# Autodesk Inventor assembly: boltAssembly
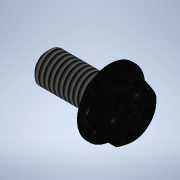
[picture p0: Inventor's stored thumbnail of the model, 180x180]
Saved by Autodesk Inventor 2020.3 (Build 243373000, 373)
## iProperties
Created: 2021-06-19
Part Number: boltAssembly
Document SubType Name: Assembly
Designer: 0x6f736f646f
Author: 0x6f736f646f
## Documents named in this file (3)
- C:\Users\Public\D\Desktop\Trash\Manufacturing-Technology-1-Project\Src\Design\boltAssembly.iam
- C:\Users\Public\D\Desktop\Trash\Manufacturing-Technology-1-Project\Src\Design\Bolt.ipt
- C:\Users\Public\D\Desktop\Trash\Manufacturing-Technology-1-Project\Src\Design\Washer.ipt
## Components (2 placed, 2 different names)
1. Bolt:1 — Mate:1, Mate:2
2. Washer:1 — Mate:1, Mate:2
## Relationships (2: Mate 2)
- Mate:1: Bolt:1 ↔ Washer:1
- Mate:2: Bolt:1 ↔ Washer:1
